# Autodesk Inventor assembly: GY81 Logger with Protoboard
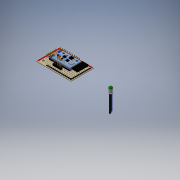
[picture p0: Inventor's stored thumbnail of the model, 180x180]
Saved by Autodesk Inventor 2016 (Build 200138000, 138)
## iProperties
Created: 2015-11-30
Part Number: GY81 Logger with Protoboard
Document SubType Name: Assembly
Designer: Spooner
Author: Spooner
## Documents named in this file (6)
- C:\Users\Spooner\Documents\GY81 Logger\3D Models\GY81 Logger with Protoboard.iam
- C:\Users\Spooner\Documents\GY81 Logger\3D Models\Arduino Pro Mini with Prog Header.iam
- C:\Users\Spooner\Documents\GY81 Logger\3D Models\Clipped LED.ipt
- C:\Users\Spooner\Documents\GY81 Logger\3D Models\G81 with Pins.iam
- C:\Users\Spooner\Documents\GY81 Logger\3D Models\MicroSD Card in Reader.iam
- C:\Users\Spooner\Documents\GY81 Logger\3D Models\Proto Board.ipt
## Components (5 placed, 5 different names)
1. Arduino Pro Mini with Prog Header:1 [sub-assembly] — Mate:4, Mate:5, Mate:6
2. Clipped LED:1
3. G81 with Pins:1 [sub-assembly] — Mate:7, Mate:8, Angle:1
4. MicroSD Card in Reader:1 [sub-assembly] — Mate:1, Mate:2, Mate:3
5. Proto Board:1 — Mate:1, Mate:2, Mate:3, Mate:4, Mate:5, Mate:6, Mate:7, Mate:8, Angle:1
## Relationships (9: Mate 8, Angle 1)
- Mate:1: MicroSD Card in Reader:1 ↔ Proto Board:1
- Mate:2: MicroSD Card in Reader:1 ↔ Proto Board:1
- Mate:3: MicroSD Card in Reader:1 ↔ Proto Board:1
- Mate:4: Arduino Pro Mini with Prog Header:1 ↔ Proto Board:1
- Mate:5: Arduino Pro Mini with Prog Header:1 ↔ Proto Board:1
- Mate:6: Arduino Pro Mini with Prog Header:1 ↔ Proto Board:1
- Mate:7: G81 with Pins:1 ↔ Proto Board:1
- Mate:8: G81 with Pins:1 ↔ Proto Board:1
- Angle:1 (0 deg): G81 with Pins:1 ↔ Proto Board:1
